# Autodesk Inventor assembly: Frame End
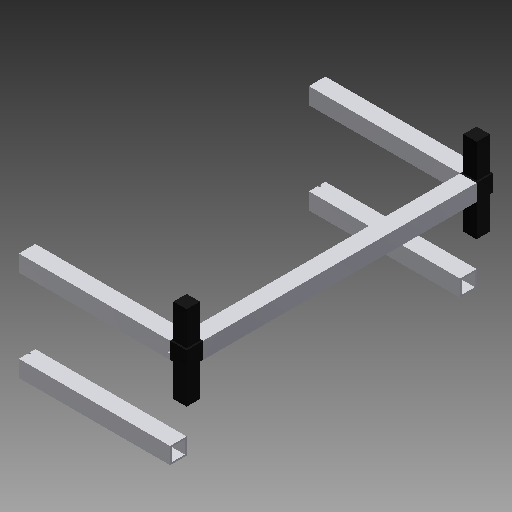
[picture p0: Inventor's stored thumbnail of the model, 512x512]
Saved by Autodesk Inventor 2017 (Build 210142000, 142)
## iProperties
Created: 2019-12-06
Part Number: Frame End
Document SubType Name: Assembly
Designer: S346553810
Author: S346553810
## Documents named in this file (4)
- \\ad.ocdsb.ca\studenthome\0\S346553810\1.Robotics\2020\2020 Robot\Frame End.iam
- \\ad.ocdsb.ca\studenthome\0\S346553810\1.Robotics\2020\2020 Robot\End cross-member.iam
- \\ad.ocdsb.ca\studenthome\0\S346553810\1.Robotics\2020\2020 Robot\1in sq tub - 10-875.ipt
- \\ad.ocdsb.ca\studenthome\0\S346553810\1.Robotics\2020\2020 Robot\End cross-member top.iam
## Components (6 placed, 3 different names)
1. End cross-member:2 [sub-assembly]
2. 1in sq tub - 10-875:1 — Flush:7, Flush:8, Flush:10
3. 1in sq tub - 10-875:2 — Flush:3, Flush:4, Mate:2, Flush:7, Flush:8, Flush:10
4. 1in sq tub - 10-875:3 — Flush:5, Flush:6, Flush:9
5. 1in sq tub - 10-875:4 — Mate:1, Flush:1, Flush:2, Flush:5, Flush:6, Flush:9
6. End cross-member top:1 [sub-assembly] — Mate:1, Flush:1, Flush:2, Flush:3, Flush:4, Mate:2
## Relationships (12: Flush 10, Mate 2)
- Mate:1: 1in sq tub - 10-875:4 ↔ End cross-member top:1
- Flush:1: 1in sq tub - 10-875:4 ↔ End cross-member top:1
- Flush:2: 1in sq tub - 10-875:4 ↔ End cross-member top:1
- Flush:3: 1in sq tub - 10-875:2 ↔ End cross-member top:1
- Flush:4: 1in sq tub - 10-875:2 ↔ End cross-member top:1
- Mate:2: 1in sq tub - 10-875:2 ↔ End cross-member top:1
- Flush:5: 1in sq tub - 10-875:3 ↔ 1in sq tub - 10-875:4
- Flush:6: 1in sq tub - 10-875:3 ↔ 1in sq tub - 10-875:4
- Flush:7: 1in sq tub - 10-875:1 ↔ 1in sq tub - 10-875:2
- Flush:8: 1in sq tub - 10-875:1 ↔ 1in sq tub - 10-875:2
- Flush:9 (-139.7 mm): 1in sq tub - 10-875:3 ↔ 1in sq tub - 10-875:4
- Flush:10 (-139.7 mm): 1in sq tub - 10-875:1 ↔ 1in sq tub - 10-875:2
